# Autodesk Inventor assembly: pcb
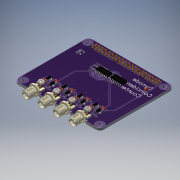
[picture p0: Inventor's stored thumbnail of the model, 180x180]
Saved by Autodesk Inventor 2016 (Build 200138000, 138)
## iProperties
Created: 2016-06-24
Part Number: pcb
Document SubType Name: Assembly
Designer: Jonathan
Author: Jonathan
## Documents named in this file (11)
- C:\Users\Jonathan\Documents\Projects\dynodePiShield\coincidenceCounter\cad\pcb.iam
- C:\Users\Jonathan\Documents\Projects\dynodePiShield\coincidenceCounter\cad\pcb.ipt
- C:\Users\Jonathan\Documents\Projects\dynodePiShield\coincidenceCounter\cad\electronics\SOT23-6.ipt
- C:\Users\Jonathan\Documents\Projects\dynodePiShield\coincidenceCounter\cad\electronics\resistor\chipResistor\chipResistor-0402.ipt
- C:\Users\Jonathan\Documents\Projects\dynodePiShield\coincidenceCounter\cad\electronics\resistor\chipResistor.ipt
- C:\Users\Jonathan\Documents\Projects\dynodePiShield\coincidenceCounter\cad\electronics\PVZ3A\PVZ3A.iam
- C:\Users\Jonathan\Documents\Projects\dynodePiShield\coincidenceCounter\cad\electronics\soic\soic-14-N.ipt
- C:\Users\Jonathan\Documents\Projects\dynodePiShield\coincidenceCounter\cad\electronics\soic\soic.ipt
- C:\Users\Jonathan\Documents\Projects\dynodePiShield\coincidenceCounter\cad\electronics\SMA Female Edge Mount CONSMA003-062.ipt
- C:\Users\Jonathan\Documents\Projects\dynodePiShield\coincidenceCounter\cad\wire.ipt
- C:\Users\Jonathan\Documents\Projects\dynodePiShield\coincidenceCounter\cad\electronics\2.54 breakaway\2x20.iam
## Components (41 placed, 8 different names)
1. pcb:1 — Mate:2, Angle:12, Mate:4, Angle:16, Mate:5, Mate:6, Mate:7, Mate:8, Mate:9, Mate:10, Angle:18, Angle:19, Angle:20, Angle:21, Angle:22, Angle:23, Angle:24, Angle:25, Mate:11, Angle:26
2. SOT23-6:1 — Flush:1, Flush:2, Flush:11, Mate:2
3. SOT23-6:2 — Flush:1, Flush:8
4. SOT23-6:3 — Flush:2, Flush:3, Flush:8, Flush:9
5. SOT23-6:4 — Flush:3, Flush:4, Flush:11, Flush:12
6. SOT23-6:5 — Flush:4, Flush:5, Flush:9, Flush:10
7. SOT23-6:6 — Flush:5, Flush:6, Flush:12, Flush:13
8. SOT23-6:7 — Flush:6, Flush:7, Flush:10
9. SOT23-6:8 — Flush:7, Flush:13
10. chipResistor-0402:3 — Flush:28, Flush:46, Mate:9
11. chipResistor-0402:4 — Flush:16, Flush:28, Flush:29, Flush:46
12. chipResistor-0402:7 — Flush:16, Flush:29, Flush:30, Flush:47
13. chipResistor-0402:10 — Flush:30, Flush:47
14. PVZ3A:1 [sub-assembly] — Angle:14, Angle:15, Flush:35, Flush:36, Flush:38, Flush:39, Mate:4
15. PVZ3A:2 [sub-assembly] — Angle:12, Angle:13, Flush:34, Flush:37
16. PVZ3A:3 [sub-assembly] — Angle:13, Angle:14, Flush:34, Flush:35, Flush:37, Flush:38
17. PVZ3A:4 [sub-assembly] — Angle:15, Flush:36, Flush:39
18. soic-14-N:1 — Angle:17, Mate:6
19. soic-14-N:2 — Angle:16, Angle:17, Mate:5
20. SMA Female Edge Mount CONSMA003-062:1 — Flush:42, Flush:45
21. SMA Female Edge Mount CONSMA003-062:2 — Flush:41, Flush:42, Flush:44, Flush:45
22. SMA Female Edge Mount CONSMA003-062:3 — Flush:40, Flush:41, Flush:43, Flush:44
23. SMA Female Edge Mount CONSMA003-062:4 — Flush:40, Flush:43, Mate:7, Mate:8
24. chipResistor-0402:11
25. chipResistor-0402:12
26. chipResistor-0402:13
27. chipResistor-0402:14
28. chipResistor-0402:15
29. chipResistor-0402:16
30. chipResistor-0402:17
31. chipResistor-0402:18
32. wire:1 — Flush:60, Flush:61, Angle:18
33. wire:2 — Flush:60, Flush:65, Mate:10, Angle:19
34. wire:3 — Flush:61, Flush:62, Angle:20
35. wire:4 — Flush:65, Flush:66, Angle:21
36. wire:5 — Flush:62, Flush:63, Angle:22
37. wire:6 — Flush:66, Flush:67, Angle:23
38. wire:7 — Flush:63, Flush:64, Angle:24
39. wire:8 — Flush:67, Angle:25
40. wire:9 — Flush:64
41. 2x20:1 [sub-assembly] — Mate:11, Angle:26
## Relationships (75: Flush 51, Angle 15, Mate 9)
- Flush:1: SOT23-6:1 ↔ SOT23-6:2
- Flush:2: SOT23-6:1 ↔ SOT23-6:3
- Flush:3: SOT23-6:3 ↔ SOT23-6:4
- Flush:4: SOT23-6:4 ↔ SOT23-6:5
- Flush:5: SOT23-6:5 ↔ SOT23-6:6
- Flush:6: SOT23-6:6 ↔ SOT23-6:7
- Flush:7: SOT23-6:7 ↔ SOT23-6:8
- Flush:8: SOT23-6:2 ↔ SOT23-6:3
- Flush:9: SOT23-6:3 ↔ SOT23-6:5
- Flush:10: SOT23-6:5 ↔ SOT23-6:7
- Flush:11: SOT23-6:1 ↔ SOT23-6:4
- Flush:12: SOT23-6:4 ↔ SOT23-6:6
- Flush:13: SOT23-6:6 ↔ SOT23-6:8
- Mate:2: pcb:1 ↔ SOT23-6:1
- Flush:16: chipResistor-0402:4 ↔ chipResistor-0402:7
- Flush:28: chipResistor-0402:3 ↔ chipResistor-0402:4
- Flush:29: chipResistor-0402:4 ↔ chipResistor-0402:7
- Flush:30: chipResistor-0402:7 ↔ chipResistor-0402:10
- Angle:12 (0 deg): pcb:1 ↔ PVZ3A:2
- Angle:13 (0 deg): PVZ3A:2 ↔ PVZ3A:3
- Angle:14 (0 deg): PVZ3A:1 ↔ PVZ3A:3
- Angle:15 (0 deg): PVZ3A:1 ↔ PVZ3A:4
- Flush:34: PVZ3A:2 ↔ PVZ3A:3
- Flush:35: PVZ3A:1 ↔ PVZ3A:3
- Flush:36: PVZ3A:1 ↔ PVZ3A:4
- Flush:37: PVZ3A:2 ↔ PVZ3A:3
- Flush:38: PVZ3A:1 ↔ PVZ3A:3
- Flush:39: PVZ3A:1 ↔ PVZ3A:4
- Mate:4: pcb:1 ↔ PVZ3A:1
- Angle:16 (0 deg): pcb:1 ↔ soic-14-N:2
- Angle:17 (0 deg): soic-14-N:1 ↔ soic-14-N:2
- Mate:5: pcb:1 ↔ soic-14-N:2
- Mate:6: pcb:1 ↔ soic-14-N:1
- Flush:40: SMA Female Edge Mount CONSMA003-062:3 ↔ SMA Female Edge Mount CONSMA003-062:4
- Flush:41: SMA Female Edge Mount CONSMA003-062:2 ↔ SMA Female Edge Mount CONSMA003-062:3
- Flush:42: SMA Female Edge Mount CONSMA003-062:1 ↔ SMA Female Edge Mount CONSMA003-062:2
- Flush:43: SMA Female Edge Mount CONSMA003-062:3 ↔ SMA Female Edge Mount CONSMA003-062:4
- Flush:44: SMA Female Edge Mount CONSMA003-062:2 ↔ SMA Female Edge Mount CONSMA003-062:3
- Flush:45: SMA Female Edge Mount CONSMA003-062:1 ↔ SMA Female Edge Mount CONSMA003-062:2
- Mate:7: pcb:1 ↔ SMA Female Edge Mount CONSMA003-062:4
- Mate:8: pcb:1 ↔ SMA Female Edge Mount CONSMA003-062:4
- Flush:46: chipResistor-0402:3 ↔ chipResistor-0402:4
- Flush:47: chipResistor-0402:7 ↔ chipResistor-0402:10
- Mate:9: pcb:1 ↔ chipResistor-0402:3
- [Flush]: chipResistor-0402:12 ↔ chipResistor-0402:13
- [Flush]: chipResistor-0402:11 ↔ chipResistor-0402:12
- [Flush]: chipResistor-0402:12 ↔ chipResistor-0402:13
- [Flush]: chipResistor-0402:13 ↔ chipResistor-0402:14
- [Flush]: chipResistor-0402:11 ↔ chipResistor-0402:12
- [Flush]: chipResistor-0402:13 ↔ chipResistor-0402:14
- [Flush]: chipResistor-0402:16 ↔ chipResistor-0402:17
- [Flush]: chipResistor-0402:15 ↔ chipResistor-0402:16
- [Flush]: chipResistor-0402:16 ↔ chipResistor-0402:17
- [Flush]: chipResistor-0402:17 ↔ chipResistor-0402:18
- [Flush]: chipResistor-0402:15 ↔ chipResistor-0402:16
- [Flush]: chipResistor-0402:17 ↔ chipResistor-0402:18
- Flush:60: wire:1 ↔ wire:2
- Flush:61: wire:1 ↔ wire:3
- Flush:62: wire:3 ↔ wire:5
- Flush:63: wire:5 ↔ wire:7
- Flush:64: wire:7 ↔ wire:9
- Flush:65: wire:2 ↔ wire:4
- Flush:66: wire:4 ↔ wire:6
- Flush:67: wire:6 ↔ wire:8
- Mate:10: pcb:1 ↔ wire:2
- Angle:18 (0 deg): pcb:1 ↔ wire:1
- Angle:19 (0 deg): pcb:1 ↔ wire:2
- Angle:20 (0 deg): pcb:1 ↔ wire:3
- Angle:21 (0 deg): pcb:1 ↔ wire:4
- Angle:22 (0 deg): pcb:1 ↔ wire:5
- Angle:23 (0 deg): pcb:1 ↔ wire:6
- Angle:24 (0 deg): pcb:1 ↔ wire:7
- Angle:25 (0 deg): pcb:1 ↔ wire:8
- Mate:11: pcb:1 ↔ 2x20:1
- Angle:26 (0 deg): pcb:1 ↔ 2x20:1
## Named parameters: d93_d90 = 0 mm, d94_d91 = 0 mm, d95_d40 = 0 mm, d96_d53 = 0 mm, d97_d54 = 0 mm, d98_d55 = 0 mm, d99_d90 = 0 mm, d100_d91 = 0 mm, d101_d40 = 0 mm, d102_d53 = 0 mm, d103_d54 = 0 mm, d104_d55 = 0 mm
